# Autodesk Inventor assembly: Swivel Arm Servo Assembly
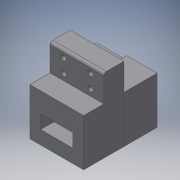
[picture p0: Inventor's stored thumbnail of the model, 180x180]
Saved by Autodesk Inventor 2019 (Build 230136000, 136)
## iProperties
Created: 2020-04-05
Part Number: Swivel Arm Servo Assembly
Document SubType Name: Assembly
Designer: isaac
Author: isaac
## Documents named in this file (3)
- C:\2_Development\Robot_arm\Swivel Arm Servo Assembly.iam
- C:\2_Development\Robot_arm\Swivel Joint Driver.ipt
- C:\2_Development\Robot_arm\LX-16A.ipt
## Components (2 placed, 2 different names)
1. Swivel Joint Driver:1 — Mate:1, Mate:2, Mate:3
2. LX-16A:1 — Mate:1, Mate:2, Mate:3
## Relationships (3: Mate 3)
- Mate:1: Swivel Joint Driver:1 ↔ LX-16A:1
- Mate:2: Swivel Joint Driver:1 ↔ LX-16A:1
- Mate:3: Swivel Joint Driver:1 ↔ LX-16A:1
